# Autodesk Inventor assembly: 合页
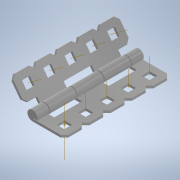
[picture p0: Inventor's stored thumbnail of the model, 180x180]
Saved by Autodesk Inventor 2020 (Build 240168000, 168)
## iProperties
Created: 2019-06-10
Part Number: 合页
Document SubType Name: Assembly
Designer: aresp
Author: aresp
## Documents named in this file (3)
- C:\Users\aresp\Documents\Vault\常用部件库\合页.iam
- C:\Users\aresp\Documents\Inventor\Content Center Files\R2020\zh-CN\合页 内\VEX Steel.ipt
- C:\Users\aresp\Documents\Inventor\Content Center Files\R2020\zh-CN\合页外\常规.ipt
## Components (2 placed, 2 different names)
1. 合页 内 VEX Steel:1 — 配合:1, 配合:2
2. 合页外 常规:1 — 配合:1, 配合:2
## Relationships (2: Mate 2)
- 配合:1 [Mate]: 合页 内 VEX Steel:1 ↔ 合页外 常规:1
- 配合:2 [Mate] (0.4064 mm): 合页 内 VEX Steel:1 ↔ 合页外 常规:1
